# Autodesk Inventor assembly: Assembly1
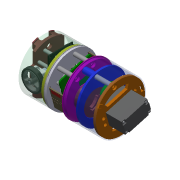
[picture p0: Inventor's stored thumbnail of the model, 180x180]
Saved by Autodesk Inventor 2018 (Build 220112000, 112)
## iProperties
Created: 2019-06-09
Part Number: Assembly1
Document SubType Name: Assembly
Designer: amink
Author: amink
## Documents named in this file (24)
- C:\Users\amink\Documents\Cad_files\tendon jaming deisgn\v1\Assembly1.iam
- C:\Users\amink\Documents\Cad_files\tendon jaming deisgn\v1\bottom_cap.ipt
- C:\Users\amink\Documents\Cad_files\tendon jaming deisgn\v1\DC_motor.ipt
- C:\Users\amink\Documents\Cad_files\tendon jaming deisgn\v1\spacer_16mm.ipt
- C:\Users\amink\Documents\Cad_files\tendon jaming deisgn\v1\pololu-wheel-32x7mm-black.ipt
- C:\Users\amink\Documents\Cad_files\tendon jaming deisgn\v1\serial_driver.ipt
- C:\Users\amink\Documents\Cad_files\tendon jaming deisgn\v1\spacer_25mm.ipt
- C:\Users\amink\Documents\Cad_files\tendon jaming deisgn\v1\base_modified_v2.ipt
- C:\Users\amink\Documents\Cad_files\tendon jaming deisgn\v1\pipe_39mm.ipt
- C:\Users\amink\Documents\Cad_files\tendon jaming deisgn\v1\base_2.ipt
- C:\Users\amink\Documents\Cad_files\tendon jaming deisgn\v1\pot.0001.ipt
- C:\Users\amink\Documents\Cad_files\tendon jaming deisgn\v1\clamp.0005.ipt
- C:\Users\amink\Documents\Cad_files\tendon jaming deisgn\v1\breadboard_spacer.ipt
- C:\Users\amink\Documents\Cad_files\tendon jaming deisgn\v1\breadbord_2_inch.ipt
- C:\Users\amink\Documents\Cad_files\tendon jaming deisgn\v1\adapter_schem.ipt
- C:\Users\amink\Documents\Cad_files\tendon jaming deisgn\v1\top_ring.ipt
- C:\Users\amink\Documents\Cad_files\tendon jaming deisgn\v1\spool\geneva_tension.ipt
- C:\Users\amink\Documents\Cad_files\tendon jaming deisgn\v1\spacer_40.ipt
- C:\Users\amink\Documents\Cad_files\tendon jaming deisgn\v1\spool\plate_r1.ipt
- C:\Users\amink\Documents\Cad_files\tendon jaming deisgn\v1\spool\top_cover_r1.ipt
- C:\Users\amink\Documents\Cad_files\tendon jaming deisgn\v1\spool\Servomoteur.ipt
- C:\Users\amink\Documents\Cad_files\tendon jaming deisgn\v1\spool\horn.ipt
- C:\Users\amink\Documents\Cad_files\tendon jaming deisgn\v1\spool\pin_r1.ipt
- C:\Users\amink\Documents\Cad_files\tendon jaming deisgn\v1\pipe_50mm.ipt
## Components (33 placed, 23 different names)
1. bottom_cap:1 — Mate:1, Mate:2, Mate:3, Mate:4, Mate:5, Mate:6, Mate:7, Mate:8, Mate:9, Mate:19, Mate:20, Mate:23
2. DC_motor:1 — Mate:1, Mate:3, Mate:4, Mate:10, Mate:11, Mate:15
3. DC_motor:2 — Mate:2, Mate:5, Mate:6, Mate:12, Mate:13, Mate:14
4. spacer_16mm:1 — Mate:7, Flush:1, Mate:17
5. spacer_16mm:2 — Mate:8, Flush:1, Mate:9, Mate:16, Mate:18
6. pololu-wheel-32x7mm-black:1 — Mate:12, Mate:13, Mate:14
7. pololu-wheel-32x7mm-black:2 — Mate:10, Mate:11, Mate:15
8. serial_driver:1 — Mate:16, Mate:17, Mate:18
9. spacer_25mm:1 — Mate:19, Mate:20, Mate:21, Mate:22
10. base_modified_v2:1 — Mate:21, Mate:22, Mate:24, Mate:25, Mate:26, Mate:27, Mate:28, Angle:1, Flush:2, Angle:2
11. pipe_39mm:1 — Mate:23, Mate:24, Mate:25
12. base_2:1 — Mate:26, Mate:29, Mate:31, Mate:32, Mate:33, Mate:34, Mate:38, Mate:39, Mate:40, Mate:41, Mate:42, Mate:43, Mate:44, Mate:45, Mate:46, Mate:47, Mate:48, Mate:49, Mate:53
13. pot.0001:1 — Mate:27, Mate:28, Angle:1, Mate:29, Mate:30
14. clamp.0005:1 — Mate:30, Flush:2, Angle:2
15. breadboard_spacer:1 — Mate:32, Mate:33, Mate:35, Mate:37
16. breadboard_spacer:2 — Mate:31, Mate:34, Mate:36
17. breadbord_2_inch:1 — Mate:35, Mate:36, Mate:37
18. adapter_schem:1 — Mate:38, Mate:39, Mate:40
19. adapter_schem:2 — Mate:41, Mate:42, Mate:43
20. top_ring:1 — Mate:52, Mate:53, Mate:54, Mate:55, Mate:56, Mate:57, Mate:58, Mate:59, Mate:62, Mate:76, Mate:78
21. spacer_25mm:2 — Mate:45, Flush:3
22. spacer_25mm:3 — Mate:44, Flush:3, Mate:49
23. spacer_25mm:4 — Mate:47, Flush:4, Mate:54
24. spacer_25mm:5 — Mate:46, Flush:4, Mate:48, Mate:52
25. geneva_tension:1 — Mate:55, Mate:76
26. spacer_40:1 — Mate:57, Mate:58, Mate:65, Mate:82, Mate:87
27. spacer_40:2 — Mate:56, Mate:59, Mate:81, Mate:86
28. plate_r1:1 — Mate:62, Mate:81, Mate:82
29. top_cover_r1:1 — Mate:65, Mate:66, Mate:74, Mate:75, Mate:77, Mate:86, Mate:87
30. Servomoteur:1 — Mate:66, Mate:69, Mate:70, Mate:74, Mate:75
31. horn:1 — Mate:69, Mate:70, Mate:71, Mate:72
32. pin_r1:1 — Mate:71, Mate:72
33. pipe_50mm:1 — Mate:77, Mate:78
## Relationships (79: Mate 73, Flush 4, Angle 2)
- Mate:1: bottom_cap:1 ↔ DC_motor:1
- Mate:2: bottom_cap:1 ↔ DC_motor:2
- Mate:3: bottom_cap:1 ↔ DC_motor:1
- Mate:4: bottom_cap:1 ↔ DC_motor:1
- Mate:5: bottom_cap:1 ↔ DC_motor:2
- Mate:6: bottom_cap:1 ↔ DC_motor:2
- Mate:7: bottom_cap:1 ↔ spacer_16mm:1
- Mate:8: bottom_cap:1 ↔ spacer_16mm:2
- Flush:1: spacer_16mm:1 ↔ spacer_16mm:2
- Mate:9: bottom_cap:1 ↔ spacer_16mm:2
- Mate:10: DC_motor:1 ↔ pololu-wheel-32x7mm-black:2
- Mate:11: DC_motor:1 ↔ pololu-wheel-32x7mm-black:2
- Mate:12: DC_motor:2 ↔ pololu-wheel-32x7mm-black:1
- Mate:13: DC_motor:2 ↔ pololu-wheel-32x7mm-black:1
- Mate:14: DC_motor:2 ↔ pololu-wheel-32x7mm-black:1
- Mate:15: DC_motor:1 ↔ pololu-wheel-32x7mm-black:2
- Mate:16: spacer_16mm:2 ↔ serial_driver:1
- Mate:17: spacer_16mm:1 ↔ serial_driver:1
- Mate:18: spacer_16mm:2 ↔ serial_driver:1
- Mate:19: bottom_cap:1 ↔ spacer_25mm:1
- Mate:20: bottom_cap:1 ↔ spacer_25mm:1
- Mate:21: spacer_25mm:1 ↔ base_modified_v2:1
- Mate:22: spacer_25mm:1 ↔ base_modified_v2:1
- Mate:23: bottom_cap:1 ↔ pipe_39mm:1
- Mate:24: base_modified_v2:1 ↔ pipe_39mm:1
- Mate:25: base_modified_v2:1 ↔ pipe_39mm:1
- Mate:26: base_modified_v2:1 ↔ base_2:1
- Mate:27: base_modified_v2:1 ↔ pot.0001:1
- Mate:28: base_modified_v2:1 ↔ pot.0001:1
- Angle:1 (0 deg): base_modified_v2:1 ↔ pot.0001:1
- Mate:29: base_2:1 ↔ pot.0001:1
- Mate:30: pot.0001:1 ↔ clamp.0005:1
- Flush:2: base_modified_v2:1 ↔ clamp.0005:1
- Angle:2 (0 deg): base_modified_v2:1 ↔ clamp.0005:1
- Mate:31: base_2:1 ↔ breadboard_spacer:2
- Mate:32: base_2:1 ↔ breadboard_spacer:1
- Mate:33: base_2:1 ↔ breadboard_spacer:1
- Mate:34: base_2:1 ↔ breadboard_spacer:2
- Mate:35: breadboard_spacer:1 ↔ breadbord_2_inch:1
- Mate:36: breadboard_spacer:2 ↔ breadbord_2_inch:1
- Mate:37: breadboard_spacer:1 ↔ breadbord_2_inch:1
- Mate:38: base_2:1 ↔ adapter_schem:1
- Mate:39: base_2:1 ↔ adapter_schem:1
- Mate:40: base_2:1 ↔ adapter_schem:1
- Mate:41: base_2:1 ↔ adapter_schem:2
- Mate:42: base_2:1 ↔ adapter_schem:2
- Mate:43: base_2:1 ↔ adapter_schem:2
- Mate:44: base_2:1 ↔ spacer_25mm:3
- Mate:45: base_2:1 ↔ spacer_25mm:2
- Mate:46: base_2:1 ↔ spacer_25mm:5
- Mate:47: base_2:1 ↔ spacer_25mm:4
- Flush:3: spacer_25mm:2 ↔ spacer_25mm:3
- Flush:4: spacer_25mm:4 ↔ spacer_25mm:5
- Mate:48: base_2:1 ↔ spacer_25mm:5
- Mate:49: base_2:1 ↔ spacer_25mm:3
- Mate:52: top_ring:1 ↔ spacer_25mm:5
- Mate:53: base_2:1 ↔ top_ring:1
- Mate:54: top_ring:1 ↔ spacer_25mm:4
- Mate:55: top_ring:1 ↔ geneva_tension:1
- Mate:56: top_ring:1 ↔ spacer_40:2
- Mate:57: top_ring:1 ↔ spacer_40:1
- Mate:58: top_ring:1 ↔ spacer_40:1
- Mate:59: top_ring:1 ↔ spacer_40:2
- Mate:62: top_ring:1 ↔ plate_r1:1
- Mate:65: spacer_40:1 ↔ top_cover_r1:1
- Mate:66: top_cover_r1:1 ↔ Servomoteur:1
- Mate:69: Servomoteur:1 ↔ horn:1
- Mate:70: Servomoteur:1 ↔ horn:1
- Mate:71: horn:1 ↔ pin_r1:1
- Mate:72: horn:1 ↔ pin_r1:1
- Mate:74: top_cover_r1:1 ↔ Servomoteur:1
- Mate:75: top_cover_r1:1 ↔ Servomoteur:1
- Mate:76: top_ring:1 ↔ geneva_tension:1
- Mate:77: top_cover_r1:1 ↔ pipe_50mm:1
- Mate:78: top_ring:1 ↔ pipe_50mm:1
- Mate:81: spacer_40:2 ↔ plate_r1:1
- Mate:82: spacer_40:1 ↔ plate_r1:1
- Mate:86: spacer_40:2 ↔ top_cover_r1:1
- Mate:87: spacer_40:1 ↔ top_cover_r1:1
